# Autodesk Inventor assembly: CL6-100
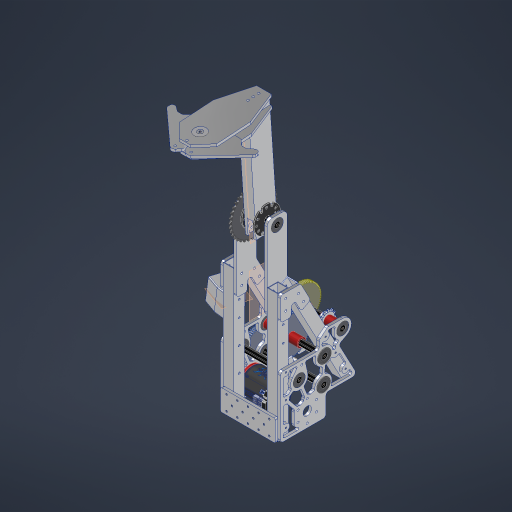
[picture p0: Inventor's stored thumbnail of the model, 512x512]
Saved by Autodesk Inventor 2023.4 (Build 274418000, 418)
## iProperties
Created: 2025-02-04
Part Number: CL6-100
Document SubType Name: Assembly
Designer: brand
Mass: 3247.43 g
Surface Area: 7567.76 cm^2
Volume: 1278.12 cm^3
Author: brand
## Documents named in this file (8)
- C:\Users\brand\OneDrive\Documents\GitHub\robotics 23\2025-ReefScape---CAD\Climber\CL6\CL6-100.iam
- C:\Users\brand\OneDrive\Documents\GitHub\robotics 23\2025-ReefScape---CAD\Climber\CL4\CL4-011.ipt
- C:\Users\brand\OneDrive\Documents\GitHub\robotics 23\2025-ReefScape---CAD\Climber\CL4\CL4-400-GB.iam
- C:\Users\brand\OneDrive\Documents\GitHub\robotics 23\2025-ReefScape---CAD\COMMON PARTS\BEARINGS\0_500_ID_x_1_125_OD_x_0_313_WD_Flanged_Bearing_217-2731.ipt
- C:\Users\brand\OneDrive\Documents\GitHub\robotics 23\2025-ReefScape---CAD\Climber\CL4\CL4-021.ipt
- C:\Users\brand\OneDrive\Documents\GitHub\robotics 23\2025-ReefScape---CAD\COMMON PARTS\ELECTRONICS\cameras\ELP Camera Angled' 17.5 + 7.5 deg up Case.ipt
- C:\Users\brand\OneDrive\Documents\GitHub\robotics 23\2025-ReefScape---CAD\Climber\CL6\CL6-200.iam
- C:\Users\brand\OneDrive\Documents\GitHub\robotics 23\2025-ReefScape---CAD\Climber\CL6\CL6-300.iam
## Components (8 placed, 7 different names)
1. CL6-200:1 [sub-assembly] — Angle:1, Insert:6, Insert:7, Insert:8, Insert:9, Insert:11, Insert:12, Insert:13, Insert:14, Flush:3
2. CL6-300:1 [sub-assembly] — Mate:2, Angle:1, Flush:3
3. CL4-011:1 — Mate:2, Mate:19, Flush:2
4. CL4-400-GB:1 [sub-assembly] — Insert:8, Insert:9
5. 0_500_ID_x_1_125_OD_x_0_313_WD_Flanged_Bearing_217-2731:1 — Insert:7
6. 0_500_ID_x_1_125_OD_x_0_313_WD_Flanged_Bearing_217-2731:2 — Insert:6, Mate:19, Flush:2
7. CL4-021:1 — Insert:11, Insert:14
8. ELP Camera Angled' 17.5 + 7.5 deg up Case:2 — Insert:12, Insert:13
## Relationships (13: Insert 8, Mate 2, Flush 2, Angle 1)
- Mate:2: CL6-300:1 ↔ CL4-011:1
- Angle:1 (0 deg): CL6-200:1 ↔ CL6-300:1
- Insert:6: CL6-200:1 ↔ 0_500_ID_x_1_125_OD_x_0_313_WD_Flanged_Bearing_217-2731:2
- Insert:7: CL6-200:1 ↔ 0_500_ID_x_1_125_OD_x_0_313_WD_Flanged_Bearing_217-2731:1
- Mate:19: CL4-011:1 ↔ 0_500_ID_x_1_125_OD_x_0_313_WD_Flanged_Bearing_217-2731:2
- Flush:2: CL4-011:1 ↔ 0_500_ID_x_1_125_OD_x_0_313_WD_Flanged_Bearing_217-2731:2
- Insert:8: CL6-200:1 ↔ CL4-400-GB:1
- Insert:9: CL6-200:1 ↔ CL4-400-GB:1
- Insert:11: CL6-200:1 ↔ CL4-021:1
- Insert:12: CL6-200:1 ↔ ELP Camera Angled' 17.5 + 7.5 deg up Case:2
- Insert:13: CL6-200:1 ↔ ELP Camera Angled' 17.5 + 7.5 deg up Case:2
- Insert:14: CL6-200:1 ↔ CL4-021:1
- Flush:3: CL6-200:1 ↔ CL6-300:1
